# Autodesk Inventor assembly: final
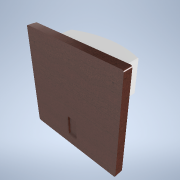
[picture p0: Inventor's stored thumbnail of the model, 180x180]
Saved by Autodesk Inventor 2021 (Build 250183000, 183)
## iProperties
Created: 2021-04-14
Part Number: final
Document SubType Name: Assembly
Designer: calst
Author: calst
## Documents named in this file (4)
- C:\Users\calst\OneDrive\Desktop\University Work\Year 3\Semester 2\Integrated Group Robotics Project\Group Task\AutoDesk Inventor\Servo\final.iam
- C:\Users\calst\OneDrive\Desktop\University Work\Year 3\Semester 2\Integrated Group Robotics Project\Group Task\AutoDesk Inventor\Board.ipt
- C:\Users\calst\OneDrive\Desktop\University Work\Year 3\Semester 2\Integrated Group Robotics Project\Group Task\AutoDesk Inventor\Servo\Twist Assembly.iam
- C:\Users\calst\OneDrive\Desktop\University Work\Year 3\Semester 2\Integrated Group Robotics Project\Group Task\AutoDesk Inventor\Playing Card RFID.ipt
## Components (3 placed, 3 different names)
1. Board:1 — Mate:1, Mate:2, Mate:3, Mate:4, Mate:5
2. Twist Assembly:1 [sub-assembly] — Mate:1, Mate:2, Mate:3
3. Playing Card RFID:1 — Mate:4, Mate:5
## Relationships (5: Mate 5)
- Mate:1: Board:1 ↔ Twist Assembly:1
- Mate:2: Board:1 ↔ Twist Assembly:1
- Mate:3: Board:1 ↔ Twist Assembly:1
- Mate:4: Board:1 ↔ Playing Card RFID:1
- Mate:5 (0.5 mm): Board:1 ↔ Playing Card RFID:1
